# Autodesk Inventor assembly: Assembled_PCB
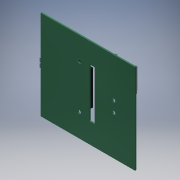
[picture p0: Inventor's stored thumbnail of the model, 180x180]
Saved by Autodesk Inventor 2017 (Build 210142000, 142)
## iProperties
Created: 2018-08-14
Part Number: Assembled_PCB
Document SubType Name: Assembly
Designer: intelsath
Author: intelsath
## Documents named in this file (14)
- C:\Users\intelsath\Documents\Inventor\Cryptowallet\Assembled_PCB.iam
- C:\Users\intelsath\Documents\Inventor\Cryptowallet\PCB.ipt
- C:\Users\intelsath\Documents\Inventor\Cryptowallet\micro_usb_connector.iam
- C:\Users\intelsath\Documents\Inventor\Cryptowallet\SiP.ipt
- C:\Users\intelsath\Documents\Inventor\Cryptowallet\RightAngleLED.ipt
- C:\Users\intelsath\Documents\Inventor\Cryptowallet\MicroSD-holder.ipt
- C:\Users\intelsath\Documents\Inventor\Cryptowallet\Pogo-pin.ipt
- C:\Users\intelsath\Documents\Inventor\Cryptowallet\Push-button.ipt
- C:\Users\intelsath\Documents\Inventor\Cryptowallet\SM02B-SRSS-TB.ipt
- C:\Users\intelsath\Documents\Inventor\Cryptowallet\LCD-Connector.ipt
- C:\Users\intelsath\Documents\Inventor\Cryptowallet\Touchscreen_Connector.ipt
- C:\Users\intelsath\Documents\Inventor\Cryptowallet\QFN32.ipt
- C:\Users\intelsath\Documents\Inventor\Cryptowallet\QFN24(4X4).ipt
- C:\Users\intelsath\Documents\Inventor\Cryptowallet\QFN-24 3x3 0.4mm.ipt
## Components (16 placed, 13 different names)
1. PCB:1 — Flush:1, Mate:1, Flush:2, Mate:2, Mate:3, Flush:3, Mate:4, Mate:5, Tangent:1, Tangent:2, Mate:6, Mate:7, Mate:8, Flush:4, Flush:5, Mate:9, Flush:6, Flush:7, Mate:10, Flush:8, Flush:9, Mate:11, Flush:10, Mate:12, Flush:11, Mate:13, Flush:12, Flush:13, Mate:14, Flush:14, Mate:15, Mate:16, Flush:15, Flush:16, Flush:17, Mate:17, Flush:18, Flush:19, Mate:18, Flush:20, Mate:19, Flush:21, Flush:22, Mate:20, Flush:23, Flush:24, Mate:21, Flush:25, Flush:26
2. micro_usb_connector:1 [sub-assembly] — Flush:1, Mate:1, Flush:2
3. SiP:1 — Mate:2, Mate:3, Tangent:1, Tangent:2
4. RightAngleLED:1 — Mate:6, Mate:7, Mate:8
5. MicroSD-holder:1 — Flush:4, Flush:5, Mate:9
6. Pogo-pin:1 — Flush:6, Flush:7, Mate:10
7. Pogo-pin:2 — Flush:8, Flush:9, Mate:11
8. Push-button:1 — Flush:10, Mate:12, Flush:11
9. SM02B-SRSS-TB:1 — Mate:13, Flush:12, Flush:13
10. LCD-Connector:1 — Mate:14, Flush:14, Mate:15
11. Touchscreen_Connector:1 — Mate:16, Flush:15, Flush:16
12. QFN32:1 — Flush:17, Mate:17, Flush:18
13. QFN32:2 — Mate:21, Flush:25, Flush:26
14. QFN24(4X4):1 — Mate:20, Flush:23, Flush:24
15. MPU-9250:1 — Mate:19, Flush:21, Flush:22
16. MPU-9250:2 — Flush:19, Mate:18, Flush:20
## Relationships (49: Flush 26, Mate 21, Tangent 2)
- Flush:1: PCB:1 ↔ micro_usb_connector:1
- Mate:1: PCB:1 ↔ micro_usb_connector:1
- Flush:2 (1.45 mm): PCB:1 ↔ micro_usb_connector:1
- Mate:2 (-17.6 mm): PCB:1 ↔ SiP:1
- Mate:3: PCB:1 ↔ SiP:1
- Flush:3: PCB:1
- Mate:4: PCB:1
- Mate:5: PCB:1
- Tangent:1: PCB:1 ↔ SiP:1
- Tangent:2: PCB:1 ↔ SiP:1
- Mate:6 (-3.1 mm): PCB:1 ↔ RightAngleLED:1
- Mate:7 (-38.9 mm): PCB:1 ↔ RightAngleLED:1
- Mate:8: PCB:1 ↔ RightAngleLED:1
- Flush:4 (1.3 mm): PCB:1 ↔ MicroSD-holder:1
- Flush:5 (1.05 mm): PCB:1 ↔ MicroSD-holder:1
- Mate:9: PCB:1 ↔ MicroSD-holder:1
- Flush:6 (6.4 mm): PCB:1 ↔ Pogo-pin:1
- Flush:7 (24.55 mm): PCB:1 ↔ Pogo-pin:1
- Mate:10: PCB:1 ↔ Pogo-pin:1
- Flush:8 (9.6 mm): PCB:1 ↔ Pogo-pin:2
- Flush:9 (24.55 mm): PCB:1 ↔ Pogo-pin:2
- Mate:11: PCB:1 ↔ Pogo-pin:2
- Flush:10 (1.66 mm): PCB:1 ↔ Push-button:1
- Mate:12: PCB:1 ↔ Push-button:1
- Flush:11 (9.6 mm): PCB:1 ↔ Push-button:1
- Mate:13: PCB:1 ↔ SM02B-SRSS-TB:1
- Flush:12 (17.84 mm): PCB:1 ↔ SM02B-SRSS-TB:1
- Flush:13 (3.06 mm): PCB:1 ↔ SM02B-SRSS-TB:1
- Mate:14: PCB:1 ↔ LCD-Connector:1
- Flush:14 (12.7 mm): PCB:1 ↔ LCD-Connector:1
- Mate:15 (-40.6 mm): PCB:1 ↔ LCD-Connector:1
- Mate:16: PCB:1 ↔ Touchscreen_Connector:1
- Flush:15 (8.15 mm): PCB:1 ↔ Touchscreen_Connector:1
- Flush:16 (19.3 mm): PCB:1 ↔ Touchscreen_Connector:1
- Flush:17 (1.35 mm): PCB:1 ↔ QFN32:1
- Mate:17: PCB:1 ↔ QFN32:1
- Flush:18 (12.05 mm): PCB:1 ↔ QFN32:1
- Flush:19 (3.2 mm): PCB:1 ↔ MPU-9250:2
- Mate:18: PCB:1 ↔ MPU-9250:2
- Flush:20 (5.9 mm): PCB:1 ↔ MPU-9250:2
- Mate:19: PCB:1 ↔ MPU-9250:1
- Flush:21 (2.05 mm): PCB:1 ↔ MPU-9250:1
- Flush:22 (27 mm): PCB:1 ↔ MPU-9250:1
- Mate:20: PCB:1 ↔ QFN24(4X4):1
- Flush:23 (2.05 mm): PCB:1 ↔ QFN24(4X4):1
- Flush:24 (32.5 mm): PCB:1 ↔ QFN24(4X4):1
- Mate:21: PCB:1 ↔ QFN32:2
- Flush:25 (16.65 mm): PCB:1 ↔ QFN32:2
- Flush:26 (5.3 mm): PCB:1 ↔ QFN32:2
